# Autodesk Inventor assembly: Bari Cart
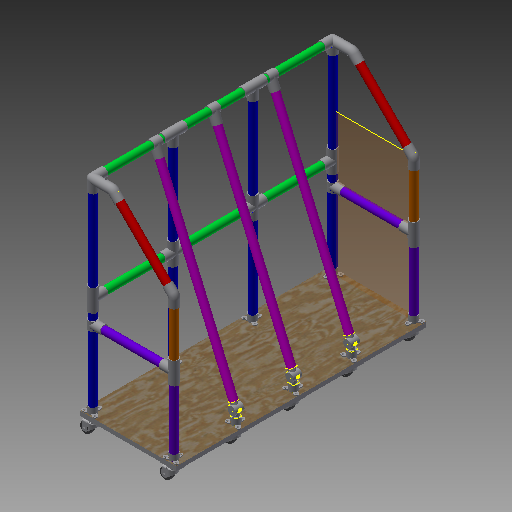
[picture p0: Inventor's stored thumbnail of the model, 512x512]
Saved by Autodesk Inventor 2018.2 (Build 222227000, 227)
## iProperties
Created: 2018-03-15
Part Number: Bari Cart
Document SubType Name: Assembly
Designer: owner
Author: owner
## Documents named in this file (18)
- Z:\The Pickle\Final Carts\Sax Cart\Bari Cart.iam
- Z:\The Pickle\Final Carts\Sax Cart\Bari Cart Base.ipt
- Z:\The Pickle\Inventor Pipe Parts\Formufit Fittings\Wood Mount 1 Inch.ipt
- Z:\The Pickle\Inventor Pipe Parts\Formufit Fittings\3-way 90 1 Inch.ipt
- Z:\The Pickle\Inventor Pipe Parts\Formufit Fittings\45 Elbow 1 Inch.ipt
- Z:\The Pickle\Inventor Pipe Parts\Formufit Fittings\Cross 1 Inch.ipt
- Z:\The Pickle\Inventor Pipe Parts\Formufit Fittings\Formufit Pipe 1 Inch Flush Fittings.ipt
- Z:\The Pickle\Inventor Pipe Parts\Formufit Fittings\Slip Tee 1 Inch.ipt
- Z:\The Pickle\Inventor Pipe Parts\Formufit Fittings\Tee 1 Inch.ipt
- Z:\The Pickle\Final Carts\Sax Cart\Adjustable Elbow 1 Inch - Sax Angle.iam
- Z:\The Pickle\Final Carts\Sax Cart\Pipe 1.ipt
- Z:\The Pickle\Final Carts\Sax Cart\Pipe 2.ipt
- Z:\The Pickle\Final Carts\Sax Cart\Pipe 3.ipt
- Z:\The Pickle\Final Carts\Sax Cart\Pipe 4.ipt
- Z:\The Pickle\Final Carts\Sax Cart\Pipe 6.ipt
- Z:\The Pickle\Final Carts\Sax Cart\Pipe 7.ipt
- Z:\The Pickle\Final Carts\Sax Cart\Pipe OD - ID adapt.ipt
- Z:\The Pickle\Final Carts\Sax Cart\Sax Wheel.ipt
## Components (72 placed, 17 different names)
1. Bari Cart Base:1 — Mate:1, Tangent:1, Tangent:2, Tangent:3, Mate:10, Mate:11, Mate:12, Flush:32, Flush:33, Flush:34, Mate:16, Tangent:4, Tangent:5, Flush:35
2. Wood Mount 1 Inch:1 — Mate:1, Tangent:1, Tangent:2, Tangent:3, Insert:1
3. Wood Mount 1 Inch:3 — Flush:3, Insert:6, Tangent:4
4. Wood Mount 1 Inch:4 — Flush:3, Flush:4, Insert:4, Tangent:5
5. Wood Mount 1 Inch:5 — Flush:5, Insert:3
6. Wood Mount 1 Inch:6 — Insert:2
7. Wood Mount 1 Inch:8 — Flush:4, Flush:5, Insert:5
8. 3-way 90 1 Inch:1 — Insert:18, Insert:21, Mate:8
9. 3-way 90 1 Inch:2 — Insert:35, Insert:37, Insert:39
10. 45 Elbow 1 Inch:1 — Insert:14
11. 45 Elbow 1 Inch:2 — Insert:42, Insert:43
12. 45 Elbow 1 Inch:3 — Insert:16, Insert:17
13. 45 Elbow 1 Inch:4 — Insert:40, Insert:41
14. Cross 1 Inch:1 — Insert:23, Insert:27, Insert:28
15. Cross 1 Inch:2 — Insert:30, Insert:31, Insert:33
16. Formufit Pipe 1 Inch Flush Fittings:1 — Insert:39, Insert:40
17. Formufit Pipe 1 Inch Flush Fittings:2 — Insert:17, Insert:18
18. Slip Tee 1 Inch:1 — Insert:12, Mate:2
19. Slip Tee 1 Inch:2 — Insert:47, Mate:3
20. Slip Tee 1 Inch:3 — Mate:6, Mate:9, Mate:15
21. Slip Tee 1 Inch:4 — Mate:5, Mate:7, Mate:9, Mate:14
22. Tee 1 Inch:1 — Insert:19, Insert:20, Insert:22
23. Tee 1 Inch:2 — Insert:36, Insert:38
24. Tee 1 Inch:3 — Insert:24, Insert:25, Insert:26
25. Tee 1 Inch:4 — Insert:29, Insert:32, Insert:34
26. Tee 1 Inch:5 — Insert:44, Insert:45, Insert:46
27. Tee 1 Inch:6 — Insert:10, Insert:11, Insert:13
28. Adjustable Elbow 1 Inch - Sax Angle:1 [sub-assembly] — Insert:53, Mate:15, Insert:56
29. Adjustable Elbow 1 Inch - Sax Angle:2 [sub-assembly] — Insert:51, Mate:13, Insert:54
30. Adjustable Elbow 1 Inch - Sax Angle:3 [sub-assembly] — Insert:52, Mate:14, Insert:55
31. Pipe 1:1 — Insert:3, Insert:31
32. Pipe 1:2 — Insert:4, Insert:38, Mate:3, Mate:23
33. Pipe 1:3 — Insert:5, Insert:28
34. Pipe 1:4 — Insert:20
35. Pipe 1:5 — Insert:25
36. Pipe 1:6 — Insert:32
37. Pipe 1:7 — Insert:37, Mate:21, Mate:22
38. Pipe 1:8 — Insert:2, Mate:2, Insert:19
39. Pipe 2:1 — Insert:21, Insert:24, Mate:4
40. Pipe 2:2 — Insert:26, Insert:29, Mate:5
41. Pipe 2:3 — Insert:33, Insert:36
42. Pipe 2:4 — Insert:34, Insert:35, Mate:6
43. Pipe 2:5 — Insert:27, Insert:30
44. Pipe 2:6 — Insert:22, Insert:23
45. Pipe 3:1 — Insert:11, Insert:12
46. Pipe 3:2 — Insert:46, Insert:47
47. Pipe 3:3 — Insert:1, Insert:10
48. Pipe 3:4 — Insert:6, Insert:45
49. Pipe 4:1 — Insert:54, Mate:17
50. Pipe 4:2 — Insert:55, Mate:18
51. Pipe 6:1 — Insert:16
52. Pipe 6:2 — Insert:41, Insert:42
53. Pipe 7:1 — Insert:13, Insert:14
54. Pipe 7:2 — Insert:43, Insert:44, Mate:20
55. Slip Tee 1 Inch:5 — Mate:4, Mate:7, Mate:8, Mate:13
56. Wood Mount 1 Inch:11 — Mate:10, Insert:50
57. Wood Mount 1 Inch:12 — Mate:11, Insert:49
58. Wood Mount 1 Inch:13 — Mate:12, Insert:48
59. Pipe OD - ID adapt:1 — Insert:48, Insert:53
60. Pipe OD - ID adapt:2 — Insert:50, Insert:51
61. Pipe OD - ID adapt:3 — Insert:49, Insert:52
62. Pipe 4:3 — Insert:56, Mate:19
63. Sax Wheel:1 — Flush:6, Flush:10, Flush:15, Flush:22, Flush:32, Flush:33
64. Sax Wheel:2 — Flush:6, Flush:7, Flush:11, Flush:16, Flush:22, Flush:23, Mate:17
65. Sax Wheel:3 — Flush:7, Flush:8, Flush:12, Flush:17, Flush:23, Flush:24, Mate:18
66. Sax Wheel:4 — Flush:8, Flush:9, Flush:13, Flush:18, Flush:24, Flush:25, Mate:19
67. Sax Wheel:5 — Flush:9, Flush:19, Flush:25, Flush:35
68. Sax Wheel:6 — Flush:14, Flush:19, Flush:27
69. Sax Wheel:7 — Flush:13, Flush:14, Flush:18, Flush:26, Flush:27
70. Sax Wheel:8 — Flush:12, Flush:17, Flush:21, Flush:26
71. Sax Wheel:9 — Flush:11, Flush:16, Flush:20, Flush:21
72. Sax Wheel:10 — Flush:10, Flush:15, Flush:20, Flush:34, Mate:16
## Relationships (111: Insert 52, Flush 29, Mate 25, Tangent 5)
- Flush:3: Wood Mount 1 Inch:3 ↔ Wood Mount 1 Inch:4
- Flush:4: Wood Mount 1 Inch:4 ↔ Wood Mount 1 Inch:8
- Flush:5: Wood Mount 1 Inch:5 ↔ Wood Mount 1 Inch:8
- Mate:1: Bari Cart Base:1 ↔ Wood Mount 1 Inch:1
- Tangent:1: Bari Cart Base:1 ↔ Wood Mount 1 Inch:1
- Tangent:2: Bari Cart Base:1 ↔ Wood Mount 1 Inch:1
- Tangent:3: Bari Cart Base:1 ↔ Wood Mount 1 Inch:1
- Insert:1: Wood Mount 1 Inch:1 ↔ Pipe 3:3
- Insert:2: Wood Mount 1 Inch:6 ↔ Pipe 1:8
- Insert:3: Wood Mount 1 Inch:5 ↔ Pipe 1:1
- Insert:4: Wood Mount 1 Inch:4 ↔ Pipe 1:2
- Insert:5: Wood Mount 1 Inch:8 ↔ Pipe 1:3
- Insert:6: Wood Mount 1 Inch:3 ↔ Pipe 3:4
- Insert:10: Tee 1 Inch:6 ↔ Pipe 3:3
- Insert:11: Tee 1 Inch:6 ↔ Pipe 3:1
- Insert:12: Slip Tee 1 Inch:1 ↔ Pipe 3:1
- Mate:2: Slip Tee 1 Inch:1 ↔ Pipe 1:8
- Insert:13: Tee 1 Inch:6 ↔ Pipe 7:1
- Insert:14: 45 Elbow 1 Inch:1 ↔ Pipe 7:1
- Insert:16: 45 Elbow 1 Inch:3 ↔ Pipe 6:1
- Insert:17: 45 Elbow 1 Inch:3 ↔ Formufit Pipe 1 Inch Flush Fittings:2
- Insert:18: 3-way 90 1 Inch:1 ↔ Formufit Pipe 1 Inch Flush Fittings:2
- Insert:19: Tee 1 Inch:1 ↔ Pipe 1:8
- Insert:20: Tee 1 Inch:1 ↔ Pipe 1:4
- Insert:21: 3-way 90 1 Inch:1 ↔ Pipe 2:1
- Insert:22: Tee 1 Inch:1 ↔ Pipe 2:6
- Insert:23: Cross 1 Inch:1 ↔ Pipe 2:6
- Insert:24: Tee 1 Inch:3 ↔ Pipe 2:1
- Insert:25: Tee 1 Inch:3 ↔ Pipe 1:5
- Insert:26: Tee 1 Inch:3 ↔ Pipe 2:2
- Insert:27: Cross 1 Inch:1 ↔ Pipe 2:5
- Insert:28: Cross 1 Inch:1 ↔ Pipe 1:3
- Insert:29: Tee 1 Inch:4 ↔ Pipe 2:2
- Insert:30: Cross 1 Inch:2 ↔ Pipe 2:5
- Insert:31: Cross 1 Inch:2 ↔ Pipe 1:1
- Insert:32: Tee 1 Inch:4 ↔ Pipe 1:6
- Insert:33: Cross 1 Inch:2 ↔ Pipe 2:3
- Insert:34: Tee 1 Inch:4 ↔ Pipe 2:4
- Insert:35: 3-way 90 1 Inch:2 ↔ Pipe 2:4
- Insert:36: Tee 1 Inch:2 ↔ Pipe 2:3
- Insert:37: 3-way 90 1 Inch:2 ↔ Pipe 1:7
- Insert:38: Tee 1 Inch:2 ↔ Pipe 1:2
- Insert:39: 3-way 90 1 Inch:2 ↔ Formufit Pipe 1 Inch Flush Fittings:1
- Insert:40: 45 Elbow 1 Inch:4 ↔ Formufit Pipe 1 Inch Flush Fittings:1
- Insert:41: 45 Elbow 1 Inch:4 ↔ Pipe 6:2
- Insert:42: 45 Elbow 1 Inch:2 ↔ Pipe 6:2
- Insert:43: 45 Elbow 1 Inch:2 ↔ Pipe 7:2
- Insert:44: Tee 1 Inch:5 ↔ Pipe 7:2
- Insert:45: Tee 1 Inch:5 ↔ Pipe 3:4
- Insert:46: Tee 1 Inch:5 ↔ Pipe 3:2
- Insert:47: Slip Tee 1 Inch:2 ↔ Pipe 3:2
- Mate:3: Slip Tee 1 Inch:2 ↔ Pipe 1:2
- Mate:4: Pipe 2:1 ↔ Slip Tee 1 Inch:5
- Mate:5: Slip Tee 1 Inch:4 ↔ Pipe 2:2
- Mate:6: Slip Tee 1 Inch:3 ↔ Pipe 2:4
- Mate:7 (225.425 mm): Slip Tee 1 Inch:4 ↔ Slip Tee 1 Inch:5
- Mate:8 (246.0625 mm): 3-way 90 1 Inch:1 ↔ Slip Tee 1 Inch:5
- Mate:9 (225.425 mm): Slip Tee 1 Inch:3 ↔ Slip Tee 1 Inch:4
- Mate:10: Bari Cart Base:1 ↔ Wood Mount 1 Inch:11
- Mate:11: Bari Cart Base:1 ↔ Wood Mount 1 Inch:12
- Mate:12: Bari Cart Base:1 ↔ Wood Mount 1 Inch:13
- Insert:48: Wood Mount 1 Inch:13 ↔ Pipe OD - ID adapt:1
- Insert:49: Wood Mount 1 Inch:12 ↔ Pipe OD - ID adapt:3
- Insert:50: Wood Mount 1 Inch:11 ↔ Pipe OD - ID adapt:2
- Insert:51: Adjustable Elbow 1 Inch - Sax Angle:2 ↔ Pipe OD - ID adapt:2
- Insert:52: Adjustable Elbow 1 Inch - Sax Angle:3 ↔ Pipe OD - ID adapt:3
- Insert:53: Adjustable Elbow 1 Inch - Sax Angle:1 ↔ Pipe OD - ID adapt:1
- Mate:13: Adjustable Elbow 1 Inch - Sax Angle:2 ↔ Slip Tee 1 Inch:5
- Mate:14: Slip Tee 1 Inch:4 ↔ Adjustable Elbow 1 Inch - Sax Angle:3
- Mate:15: Slip Tee 1 Inch:3 ↔ Adjustable Elbow 1 Inch - Sax Angle:1
- Insert:54: Adjustable Elbow 1 Inch - Sax Angle:2 ↔ Pipe 4:1
- Insert:55: Adjustable Elbow 1 Inch - Sax Angle:3 ↔ Pipe 4:2
- Insert:56: Adjustable Elbow 1 Inch - Sax Angle:1 ↔ Pipe 4:3
- Flush:6: Sax Wheel:1 ↔ Sax Wheel:2
- Flush:7: Sax Wheel:2 ↔ Sax Wheel:3
- Flush:8: Sax Wheel:3 ↔ Sax Wheel:4
- Flush:9: Sax Wheel:4 ↔ Sax Wheel:5
- Flush:10: Sax Wheel:1 ↔ Sax Wheel:10
- Flush:11: Sax Wheel:2 ↔ Sax Wheel:9
- Flush:12: Sax Wheel:3 ↔ Sax Wheel:8
- Flush:13: Sax Wheel:4 ↔ Sax Wheel:7
- Flush:14: Sax Wheel:6 ↔ Sax Wheel:7
- Flush:15: Sax Wheel:1 ↔ Sax Wheel:10
- Flush:16: Sax Wheel:2 ↔ Sax Wheel:9
- Flush:17: Sax Wheel:3 ↔ Sax Wheel:8
- Flush:18: Sax Wheel:4 ↔ Sax Wheel:7
- Flush:19: Sax Wheel:5 ↔ Sax Wheel:6
- Flush:20: Sax Wheel:9 ↔ Sax Wheel:10
- Flush:21: Sax Wheel:8 ↔ Sax Wheel:9
- Flush:22: Sax Wheel:1 ↔ Sax Wheel:2
- Flush:23: Sax Wheel:2 ↔ Sax Wheel:3
- Flush:24: Sax Wheel:3 ↔ Sax Wheel:4
- Flush:25: Sax Wheel:4 ↔ Sax Wheel:5
- Flush:26: Sax Wheel:7 ↔ Sax Wheel:8
- Flush:27: Sax Wheel:6 ↔ Sax Wheel:7
- Flush:32: Bari Cart Base:1 ↔ Sax Wheel:1
- Flush:33: Bari Cart Base:1 ↔ Sax Wheel:1
- Flush:34: Bari Cart Base:1 ↔ Sax Wheel:10
- Mate:16: Bari Cart Base:1 ↔ Sax Wheel:10
- Mate:17 (-22.225 mm): Pipe 4:1 ↔ Sax Wheel:2
- Mate:18 (-22.225 mm): Pipe 4:2 ↔ Sax Wheel:3
- Mate:19 (-22.225 mm): Pipe 4:3 ↔ Sax Wheel:4
- Tangent:4: Bari Cart Base:1 ↔ Wood Mount 1 Inch:3
- Tangent:5: Bari Cart Base:1 ↔ Wood Mount 1 Inch:4
- Flush:35: Bari Cart Base:1 ↔ Sax Wheel:5
- Mate:20: Pipe 7:2
- Mate:21: Pipe 1:7
- Mate:22: Pipe 1:7
- Mate:23: Pipe 1:2
- Mate:24
- Mate:25
